# Autodesk Inventor assembly: DPLX_A001_revE_Electrode_assmMJS
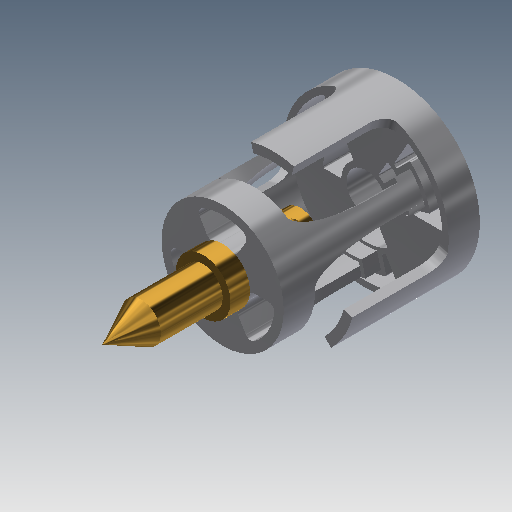
[picture p0: Inventor's stored thumbnail of the model, 512x512]
Saved by Autodesk Inventor 2018 (Build 220112000, 112)
## iProperties
Created: 2018-03-16
Part Number: DPLX_A001_revE_Electrode_assmMJS
Document SubType Name: Assembly
Designer: DPLXuser
Sending System: SolidWorks 2017
Last Author: Dplxuser
Last Saved: 2018-04-10
Author: DPLXuser
## Documents named in this file (5)
- C:\Users\DPLXuser\Documents\GitHub\UMBC_DPLX_SPARK\SPARK CAD Files\DPLX_A001_revE_Electrode_assmMJS.iam
- C:\Users\DPLXuser\Documents\GitHub\UMBC_DPLX_SPARK\SPARK CAD Files\DPLX_P004_revD_large_outside_baffle.ipt
- C:\Users\DPLXuser\Documents\GitHub\UMBC_DPLX_SPARK\SPARK CAD Files\DPLX_P001_Electrode.ipt
- C:\Users\DPLXuser\Documents\GitHub\UMBC_DPLX_SPARK\SPARK CAD Files\DPLX_P006_BRASS SOCKET HEAD CAP SCREW.ipt
- C:\Users\DPLXuser\Documents\GitHub\UMBC_DPLX_SPARK\SPARK CAD Files\DPLX_P003_small_inside_baffle_RevB.ipt
## Components (4 placed, 4 different names)
1. DPLX_P001_Electrode:1 — Mate:1, Mate:2, Insert:1, Insert:2
2. DPLX_P006_BRASS SOCKET HEAD CAP SCREW:1 — Mate:1, Mate:2
3. DPLX_P003_small_inside_baffle_RevB:1 — Insert:1
4. DPLX_P004_revD_large_outside_baffle:1 — Insert:2
## Relationships (4: Mate 2, Insert 2)
- Mate:1: DPLX_P001_Electrode:1 ↔ DPLX_P006_BRASS SOCKET HEAD CAP SCREW:1
- Mate:2: DPLX_P001_Electrode:1 ↔ DPLX_P006_BRASS SOCKET HEAD CAP SCREW:1
- Insert:1: DPLX_P001_Electrode:1 ↔ DPLX_P003_small_inside_baffle_RevB:1
- Insert:2 (-15.748 mm): DPLX_P001_Electrode:1 ↔ DPLX_P004_revD_large_outside_baffle:1
